# Autodesk Inventor assembly: tip2_ass_t2
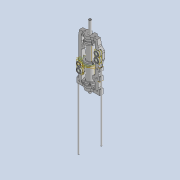
[picture p0: Inventor's stored thumbnail of the model, 180x180]
Saved by Autodesk Inventor 2020 (Build 240168000, 168)
## iProperties
Created: 2021-07-21
Part Number: tip2_ass_t2
Document SubType Name: Assembly
Designer: Shuang Peng
Author: Shuang Peng
## Documents named in this file (7)
- D:\projects-3\torque fb tip\hardware\tip_2\tip2_ass_t2.iam
- D:\projects-3\torque fb tip\hardware\tip_2\cable_holder_2.ipt
- D:\projects-3\torque fb tip\hardware\tip_2\bearing_3_6_2.ipt
- D:\projects-3\torque fb tip\hardware\tip_2\bearing_holder_2.ipt
- D:\projects-3\torque fb tip\hardware\tip_2\bw_tube_2.ipt
- D:\projects-3\torque fb tip\hardware\tip_2\cab_coil_smooth.ipt
- D:\projects-3\torque fb tip\hardware\tip_2\pin_3_40.ipt
## Components (19 placed, 6 different names)
1. cable_holder_2:1 — Insert:1, Insert:2, Insert:5, Insert:6, Insert:11, Insert:12, Insert:13, Insert:14, Insert:15, Insert:16
2. bearing_3_6_2:1 — Insert:2, Insert:4
3. bearing_3_6_2:2 — Insert:3
4. bearing_3_6_2:3 — Insert:4
5. bearing_3_6_2:4 — Insert:1, Insert:3
6. bearing_3_6_2:5 — Insert:5, Insert:7
7. bearing_3_6_2:6 — Insert:6, Insert:8
8. bearing_3_6_2:7 — Insert:7
9. bearing_3_6_2:8 — Insert:8
10. bearing_holder_2:1 — Insert:9, Insert:11, Insert:12
11. bearing_holder_2:2 — Insert:10, Insert:13, Insert:14
12. bearing_3_6_2:9 — Insert:9
13. bearing_3_6_2:10 — Insert:10, Insert:20
14. bw_tube_2:1 — Insert:15
15. bw_tube_2:2 — Insert:16
16. cab_coil_smooth:1 — Insert:17, Insert:19, Insert:20
17. cab_coil_smooth:2 — Insert:17, Insert:18
18. pin_3_40:1 — Insert:18
19. pin_3_40:2 — Insert:19
## Relationships (20: Insert 20)
- Insert:1: cable_holder_2:1 ↔ bearing_3_6_2:4
- Insert:2: cable_holder_2:1 ↔ bearing_3_6_2:1
- Insert:3: bearing_3_6_2:2 ↔ bearing_3_6_2:4
- Insert:4: bearing_3_6_2:1 ↔ bearing_3_6_2:3
- Insert:5: cable_holder_2:1 ↔ bearing_3_6_2:5
- Insert:6: cable_holder_2:1 ↔ bearing_3_6_2:6
- Insert:7: bearing_3_6_2:5 ↔ bearing_3_6_2:7
- Insert:8: bearing_3_6_2:6 ↔ bearing_3_6_2:8
- Insert:9: bearing_holder_2:1 ↔ bearing_3_6_2:9
- Insert:10: bearing_holder_2:2 ↔ bearing_3_6_2:10
- Insert:11: cable_holder_2:1 ↔ bearing_holder_2:1
- Insert:12: cable_holder_2:1 ↔ bearing_holder_2:1
- Insert:13: cable_holder_2:1 ↔ bearing_holder_2:2
- Insert:14: cable_holder_2:1 ↔ bearing_holder_2:2
- Insert:15: cable_holder_2:1 ↔ bw_tube_2:1
- Insert:16: cable_holder_2:1 ↔ bw_tube_2:2
- Insert:17: cab_coil_smooth:1 ↔ cab_coil_smooth:2
- Insert:18 (-20 mm): cab_coil_smooth:2 ↔ pin_3_40:1
- Insert:19 (-30 mm): cab_coil_smooth:1 ↔ pin_3_40:2
- Insert:20 (0.5 mm): bearing_3_6_2:10 ↔ cab_coil_smooth:1
